# Autodesk Inventor assembly: Assembly4
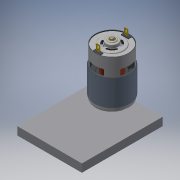
[picture p0: Inventor's stored thumbnail of the model, 180x180]
Saved by Autodesk Inventor 2019.4 (Build 234330000, 330)
## iProperties
Created: 2020-04-12
Part Number: Assembly4
Document SubType Name: Assembly
Designer: Niran
Author: Niran
## Documents named in this file (3)
- C:\Users\Niran\Desktop\sketch_jan26a\Canon parts\Assembly4.iam
- C:\Users\Niran\Desktop\sketch_jan26a\Canon parts\Part40.ipt
- C:\Users\Niran\Desktop\sketch_jan26a\Canon parts\DC Motor.ipt
## Components (2 placed, 2 different names)
1. Part40:1 — Rigid:1
2. DC Motor:1 — Rigid:1
## Relationships (1: WeldJoint 1)
- Rigid:1 [WeldJoint] (-6 mm): Part40:1 ↔ DC Motor:1
